# Autodesk Inventor assembly: 2h
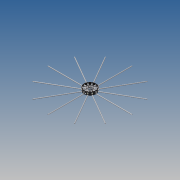
[picture p0: Inventor's stored thumbnail of the model, 180x180]
Saved by Autodesk Inventor 2014 SP1 (Build 180222100, 222)
## iProperties
Created: 2013-12-02
Part Number: 2h
Document SubType Name: Assembly
Designer: Dave
Description: Hub
Author: Dave
## Documents named in this file (11)
- C:\Users\Dave\Desktop\hera-cad\hub\hub.iam
- C:\Users\Dave\Desktop\hera-cad\hub\sonotubeInner.ipt
- C:\Users\Dave\Desktop\hera-cad\hub\sonotubeOuter.ipt
- C:\Users\Dave\Desktop\hera-cad\hub\conduit.ipt
- C:\Users\Dave\Desktop\hera-cad\hub\rebarbar.ipt
- C:\Users\Dave\Desktop\hera-cad\hub\rebarcircle.ipt
- C:\Users\Dave\Desktop\hera-cad\hub\cement.ipt
- C:\Users\Dave\Desktop\hera-cad\hub\sleeve_spar.ipt
- C:\Users\Dave\Desktop\hera-cad\hub\hubVertRebar.ipt
- C:\Users\Dave\Desktop\hera-cad\support\sparHoriz.ipt
- C:\Users\Dave\Desktop\hera-cad\smallParts\nail_20d.ipt
## Components (81 placed, 10 different names)
1. sonotubeInner:1 — Insert:1, Insert:2, Insert:5, Angle:3
2. sonotubeOuter:1 — Insert:1, Mate:3, Insert:6, Insert:7
3. rebarbar:1 — Insert:5
4. rebarcircle:1
5. cement:1 — Insert:2
6. conduit:1
7. hubVertRebar:2
8. hubVertRebar:3
9. hubVertRebar:4
10. sparHoriz:1 — Insert:7, Angle:1, Angle:2, Angle:3, Mate:4, Mate:5
11. nail_20d:1 — Angle:1, Mate:4
12. nail_20d:2 — Angle:2, Mate:5
13. sparHoriz:2
14. nail_20d:3
15. nail_20d:4
16. sparHoriz:3
17. nail_20d:5
18. nail_20d:6
19. sparHoriz:4
20. nail_20d:7
21. nail_20d:8
22. sparHoriz:5
23. nail_20d:9
24. nail_20d:10
25. sparHoriz:6
26. nail_20d:11
27. nail_20d:12
28. sparHoriz:7
29. nail_20d:13
30. nail_20d:14
31. sparHoriz:8
32. nail_20d:15
33. nail_20d:16
34. sparHoriz:9
35. nail_20d:17
36. nail_20d:18
37. sparHoriz:10
38. nail_20d:19
39. nail_20d:20
40. sparHoriz:11
41. nail_20d:21
42. nail_20d:22
43. sparHoriz:12
44. nail_20d:23
45. nail_20d:24
46. sleeve_spar:1 — Mate:3, Insert:6, Angle:4, Mate:6, Angle:5, Mate:7
47. nail_20d:26 — Angle:5, Mate:7
48. nail_20d:25 — Angle:4, Mate:6
49. sleeve_spar:2
50. nail_20d:27
51. nail_20d:28
52. sleeve_spar:3
53. nail_20d:29
54. nail_20d:30
55. sleeve_spar:4
56. nail_20d:31
57. nail_20d:32
58. sleeve_spar:5
59. nail_20d:33
60. nail_20d:34
61. sleeve_spar:6
62. nail_20d:35
63. nail_20d:36
64. sleeve_spar:7
65. nail_20d:37
66. nail_20d:38
67. sleeve_spar:8
68. nail_20d:39
69. nail_20d:40
70. sleeve_spar:9
71. nail_20d:41
72. nail_20d:42
73. sleeve_spar:10
74. nail_20d:43
75. nail_20d:44
76. sleeve_spar:11
77. nail_20d:45
78. nail_20d:46
79. sleeve_spar:12
80. nail_20d:47
81. nail_20d:48
## Component patterns: vertRebar (3 elements), supportHoriz (12 elements), (12 elements, first: sleeve_spar:1 + nail_20d:26 + nail_20d:25)
## Relationships (15: Insert 5, Mate 5, Angle 5)
- Insert:1: sonotubeInner:1 ↔ sonotubeOuter:1
- Insert:2: sonotubeInner:1 ↔ cement:1
- Insert:5 (-101.6 mm): sonotubeInner:1 ↔ rebarbar:1
- Mate:3: sonotubeOuter:1 ↔ sleeve_spar:1
- Insert:6 (-271.78 mm): sonotubeOuter:1 ↔ sleeve_spar:1
- Insert:7 (-266.7 mm): sonotubeOuter:1 ↔ sparHoriz:1
- Angle:1 (180 deg): sparHoriz:1 ↔ nail_20d:1
- Angle:2 (180 deg): sparHoriz:1 ↔ nail_20d:2
- Angle:3 (180 deg): sonotubeInner:1 ↔ sparHoriz:1
- Mate:4: sparHoriz:1 ↔ nail_20d:1
- Mate:5: sparHoriz:1 ↔ nail_20d:2
- Angle:4 (180 deg): sleeve_spar:1 ↔ nail_20d:25
- Mate:6: sleeve_spar:1 ↔ nail_20d:25
- Angle:5 (180 deg): sleeve_spar:1 ↔ nail_20d:26
- Mate:7: sleeve_spar:1 ↔ nail_20d:26
